# Autodesk Inventor assembly: layout
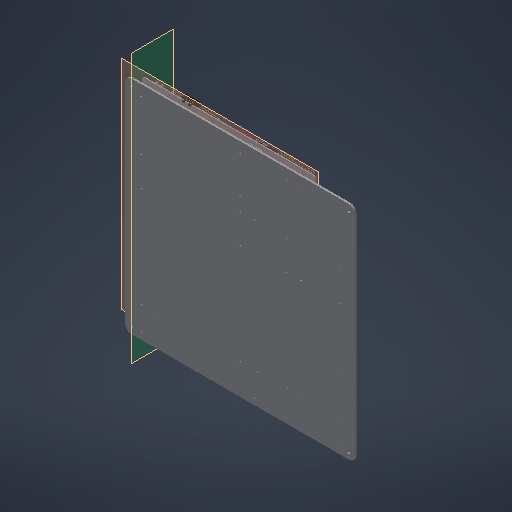
[picture p0: Inventor's stored thumbnail of the model, 512x512]
Saved by Autodesk Inventor 2026 (Build 300175000, 175)
## iProperties
Created: 2019-10-14
Part Number: layout
Material: 一般
Document SubType Name: Assembly
Designer: gisen
Author: gisen
## Documents named in this file (5)
- C:\Users\numai\Documents\workspace\inventor\eatx_case\robocup\layout.iam
- C:\Users\numai\Documents\workspace\inventor\eatx_case\eatx_slim\resources\motherboard\Rampage V Extreme Assembly.iam
- C:\Users\numai\Documents\workspace\inventor\eatx_case\robocup\mb_plate_01.ipt
- C:\Users\numai\Documents\workspace\inventor\eatx_case\robocup\io_fix.ipt
- C:\Users\numai\Documents\workspace\inventor\eatx_case\robocup\spacer.ipt
## Components (4 placed, 4 different names)
1. Rampage V Extreme Assembly:1 [sub-assembly] — フラッシュ:1, メイト:2, メイト:4
2. mb_plate_01:1 — メイト:1, メイト:3
3. io_fix:1 — フラッシュ:2
4. spacer:1 — メイト:3, メイト:4
## Relationships (7: Mate 4, Flush 2, Angle 1)
- フラッシュ:1 [Flush] (8 mm): Rampage V Extreme Assembly:1
- メイト:1 [Mate]: mb_plate_01:1
- メイト:2 [Mate]: Rampage V Extreme Assembly:1
- 角度:1 [Angle] (0 deg)
- フラッシュ:2 [Flush]: io_fix:1
- メイト:3 [Mate]: mb_plate_01:1 ↔ spacer:1
- メイト:4 [Mate]: Rampage V Extreme Assembly:1 ↔ spacer:1
